# Autodesk Inventor assembly: field
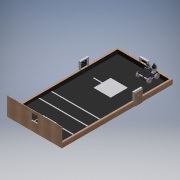
[picture p0: Inventor's stored thumbnail of the model, 180x180]
Saved by Autodesk Inventor 2017 (Build 210142000, 142)
## iProperties
Created: 2016-12-21
Part Number: field
Document SubType Name: Assembly
Designer: Naga
Author: Naga
## Documents named in this file (19)
- E:\GDrive\IEEE CS\SoutheastCon2017\Cad\Field\field.iam
- E:\GDrive\IEEE CS\SoutheastCon2017\Cad\Field\wallLeftLong.ipt
- E:\GDrive\IEEE CS\SoutheastCon2017\Cad\Field\wallLeftShort.ipt
- E:\GDrive\IEEE CS\SoutheastCon2017\Cad\Field\wallRightLong.ipt
- E:\GDrive\IEEE CS\SoutheastCon2017\Cad\Field\wallRightShort.ipt
- E:\GDrive\IEEE CS\SoutheastCon2017\Cad\Field\baseField.ipt
- E:\GDrive\IEEE CS\SoutheastCon2017\Cad\Field\backBoard.ipt
- E:\GDrive\IEEE CS\SoutheastCon2017\Cad\Field\shootFrame.ipt
- E:\GDrive\IEEE CS\SoutheastCon2017\Cad\Field\floorLayer.ipt
- E:\GDrive\IEEE CS\SoutheastCon2017\Cad\Field\floorTopLayer.ipt
- E:\GDrive\IEEE CS\SoutheastCon2017\Cad\Field\floorMidLayer.ipt
- E:\GDrive\IEEE CS\SoutheastCon2017\Cad\Field\topStair.ipt
- E:\GDrive\IEEE CS\SoutheastCon2017\Cad\Field\Stage1Wall.ipt
- E:\GDrive\IEEE CS\SoutheastCon2017\Cad\Field\Stage2Wall.ipt
- E:\GDrive\IEEE CS\SoutheastCon2017\Cad\Field\Stage3Wall.ipt
- E:\GDrive\IEEE CS\SoutheastCon2017\Cad\Field\sideStage2Frame.ipt
- E:\GDrive\IEEE CS\SoutheastCon2017\Cad\Field\sideStage13Frame.ipt
- E:\GDrive\IEEE CS\SoutheastCon2017\Cad\Field\topStageFrame.ipt
- E:\GDrive\IEEE CS\SoutheastCon2017\Cad\completeRobot.iam
## Components (27 placed, 18 different names)
1. wallLeftLong:1 — Mate:1, Mate:2, Mate:3, Mate:4, Mate:5, Mate:6, Mate:7, Mate:8, Mate:13, Flush:1, Flush:6, Mate:29, Mate:36, Flush:25, Mate:45, Mate:46, Flush:33, Flush:34
2. wallLeftShort:1 — Mate:3, Mate:4, Mate:5, Flush:2, Mate:21, Mate:34
3. wallRightLong:1 — Mate:9, Mate:10, Mate:11, Mate:37, Mate:40
4. wallRightShort:1 — Mate:6, Mate:7, Mate:8, Mate:9, Mate:10, Mate:11, Mate:12, Flush:23, Mate:35, Flush:24, Flush:28, Mate:50, Flush:39
5. baseField:1 — Mate:13, Flush:1, Flush:2, Flush:5, Mate:28, Mate:32, Flush:52
6. backBoard:1 — Flush:3, Flush:4, Mate:20, Mate:21, Flush:5, Flush:6
7. shootFrame:1 — Mate:14, Mate:15
8. shootFrame:2 — Mate:15, Mate:18, Mate:19, Flush:4, Mate:20
9. shootFrame:3 — Mate:16, Mate:17, Mate:18, Mate:19, Flush:3
10. shootFrame:4 — Mate:14, Mate:16, Mate:17
11. floorLayer:2 — Mate:25, Mate:28, Mate:32, Flush:18, Flush:19
12. floorTopLayer:4 — Flush:13, Flush:17, Mate:31, Flush:20, Flush:21, Mate:33, Flush:22
13. floorMidLayer:2 — Mate:25, Flush:13, Mate:29, Flush:18, Flush:19, Flush:20, Flush:21, Mate:33
14. topStair:1 — Flush:17, Mate:31, Flush:22, Mate:34
15. Stage1Wall:1 — Flush:26, Flush:27, Mate:37, Mate:38, Mate:39, Mate:41
16. Stage2Wall:1 — Flush:23, Mate:35, Flush:24, Mate:43, Mate:48
17. Stage3Wall:1 — Mate:36, Flush:25, Flush:26, Flush:27, Flush:28, Mate:44, Mate:47
18. sideStage2Frame:1 — Mate:48, Mate:49, Flush:38, Flush:41, Mate:51
19. sideStage13Frame:1 — Flush:29, Flush:30, Mate:41, Flush:31, Flush:32
20. topStageFrame:1 — Mate:43, Mate:49, Flush:40, Flush:41, Flush:42
21. sideStage2Frame:2 — Mate:50, Flush:38, Flush:39, Flush:40, Flush:42
22. sideStage13Frame:2 — Mate:46, Flush:33, Flush:35, Flush:37
23. topStageFrame:2 — Mate:44, Flush:34, Flush:36, Flush:37
24. topStageFrame:3 — Mate:42, Flush:31, Flush:32
25. sideStage13Frame:3 — Mate:45, Flush:35, Flush:36, Mate:47
26. sideStage13Frame:4 — Mate:38, Mate:39, Mate:40, Flush:29, Flush:30, Mate:42
27. completeRobot:1 [sub-assembly] — Flush:52, Mate:51
## Relationships (79: Mate 45, Flush 34)
- Mate:1: wallLeftLong:1
- Mate:2: wallLeftLong:1
- Mate:3: wallLeftLong:1 ↔ wallLeftShort:1
- Mate:4: wallLeftLong:1 ↔ wallLeftShort:1
- Mate:5: wallLeftLong:1 ↔ wallLeftShort:1
- Mate:6: wallLeftLong:1 ↔ wallRightShort:1
- Mate:7: wallLeftLong:1 ↔ wallRightShort:1
- Mate:8: wallLeftLong:1 ↔ wallRightShort:1
- Mate:9: wallRightLong:1 ↔ wallRightShort:1
- Mate:10: wallRightLong:1 ↔ wallRightShort:1
- Mate:11: wallRightLong:1 ↔ wallRightShort:1
- Mate:12: wallRightShort:1
- Mate:13: wallLeftLong:1 ↔ baseField:1
- Flush:1: wallLeftLong:1 ↔ baseField:1
- Flush:2: wallLeftShort:1 ↔ baseField:1
- Mate:14: shootFrame:1 ↔ shootFrame:4
- Mate:15: shootFrame:1 ↔ shootFrame:2
- Mate:16: shootFrame:3 ↔ shootFrame:4
- Mate:17: shootFrame:3 ↔ shootFrame:4
- Mate:18: shootFrame:2 ↔ shootFrame:3
- Mate:19: shootFrame:2 ↔ shootFrame:3
- Flush:3: backBoard:1 ↔ shootFrame:3
- Flush:4: backBoard:1 ↔ shootFrame:2
- Mate:20: backBoard:1 ↔ shootFrame:2
- Mate:21: wallLeftShort:1 ↔ backBoard:1
- Flush:5: baseField:1 ↔ backBoard:1
- Flush:6: wallLeftLong:1 ↔ backBoard:1
- Mate:25: floorLayer:2 ↔ floorMidLayer:2
- Flush:13: floorTopLayer:4 ↔ floorMidLayer:2
- Mate:28: baseField:1 ↔ floorLayer:2
- Mate:29: wallLeftLong:1 ↔ floorMidLayer:2
- Flush:17: floorTopLayer:4 ↔ topStair:1
- Mate:31: floorTopLayer:4 ↔ topStair:1
- Mate:32: baseField:1 ↔ floorLayer:2
- Flush:18: floorLayer:2 ↔ floorMidLayer:2
- Flush:19: floorLayer:2 ↔ floorMidLayer:2
- Flush:20: floorTopLayer:4 ↔ floorMidLayer:2
- Flush:21: floorTopLayer:4 ↔ floorMidLayer:2
- Mate:33: floorTopLayer:4 ↔ floorMidLayer:2
- Flush:22 (419.1 mm): floorTopLayer:4 ↔ topStair:1
- Mate:34: wallLeftShort:1 ↔ topStair:1
- Flush:23 (-76.2 mm): wallRightShort:1 ↔ Stage2Wall:1
- Mate:35: wallRightShort:1 ↔ Stage2Wall:1
- Flush:24 (533.4 mm): wallRightShort:1 ↔ Stage2Wall:1
- Mate:36: wallLeftLong:1 ↔ Stage3Wall:1
- Flush:25 (-152.4 mm): wallLeftLong:1 ↔ Stage3Wall:1
- Flush:26: Stage1Wall:1 ↔ Stage3Wall:1
- Flush:27: Stage1Wall:1 ↔ Stage3Wall:1
- Mate:37: wallRightLong:1 ↔ Stage1Wall:1
- Flush:28 (685.8 mm): wallRightShort:1 ↔ Stage3Wall:1
- Mate:38: Stage1Wall:1 ↔ sideStage13Frame:4
- Mate:39: Stage1Wall:1 ↔ sideStage13Frame:4
- Mate:40: wallRightLong:1 ↔ sideStage13Frame:4
- Flush:29: sideStage13Frame:1 ↔ sideStage13Frame:4
- Flush:30: sideStage13Frame:1 ↔ sideStage13Frame:4
- Mate:41: Stage1Wall:1 ↔ sideStage13Frame:1
- Mate:42: topStageFrame:3 ↔ sideStage13Frame:4
- Flush:31: sideStage13Frame:1 ↔ topStageFrame:3
- Flush:32: sideStage13Frame:1 ↔ topStageFrame:3
- Mate:43: Stage2Wall:1 ↔ topStageFrame:1
- Mate:44: Stage3Wall:1 ↔ topStageFrame:2
- Mate:45: wallLeftLong:1 ↔ sideStage13Frame:3
- Mate:46: wallLeftLong:1 ↔ sideStage13Frame:2
- Flush:33: wallLeftLong:1 ↔ sideStage13Frame:2
- Flush:34: wallLeftLong:1 ↔ topStageFrame:2
- Flush:35: sideStage13Frame:2 ↔ sideStage13Frame:3
- Flush:36: topStageFrame:2 ↔ sideStage13Frame:3
- Flush:37: sideStage13Frame:2 ↔ topStageFrame:2
- Mate:47: Stage3Wall:1 ↔ sideStage13Frame:3
- Mate:48: Stage2Wall:1 ↔ sideStage2Frame:1
- Mate:49: sideStage2Frame:1 ↔ topStageFrame:1
- Mate:50: wallRightShort:1 ↔ sideStage2Frame:2
- Flush:38: sideStage2Frame:1 ↔ sideStage2Frame:2
- Flush:39: wallRightShort:1 ↔ sideStage2Frame:2
- Flush:40: topStageFrame:1 ↔ sideStage2Frame:2
- Flush:41: sideStage2Frame:1 ↔ topStageFrame:1
- Flush:42: topStageFrame:1 ↔ sideStage2Frame:2
- Flush:52: baseField:1 ↔ completeRobot:1
- Mate:51: sideStage2Frame:1 ↔ completeRobot:1
